# Autodesk Inventor assembly: rodAndKey
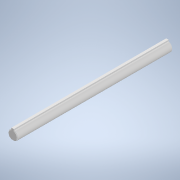
[picture p0: Inventor's stored thumbnail of the model, 180x180]
Saved by Autodesk Inventor 2020.2 (Build 242310000, 310)
## iProperties
Created: 2019-12-09
Part Number: rodAndKey
Document SubType Name: Assembly
Designer: robst
Author: robst
## Documents named in this file (3)
- C:\git\CAD-Development\robSteele\liftSpool\rodAndKey.iam
- C:\git\CAD-Development\robSteele\liftSpool\6 inch 98491A098_OVERSIZED STEEL MACHINE KEY STOCK.ipt
- C:\git\CAD-Development\robSteele\liftSpool\6 inch 1570K330_FULLY KEYED ALUMINUM DRIVE SHAFT.ipt
## Components (2 placed, 2 different names)
1. 6 inch 1570K330_FULLY KEYED ALUMINUM DRIVE SHAFT:1
2. 6 inch 98491A098_OVERSIZED STEEL MACHINE KEY STOCK:1
## Relationships (2: Mate 1, Flush 1)
- [Mate]: 6 inch 1570K330_FULLY KEYED ALUMINUM DRIVE SHAFT:1 ↔ 6 inch 98491A098_OVERSIZED STEEL MACHINE KEY STOCK:1
- [Flush]: 6 inch 1570K330_FULLY KEYED ALUMINUM DRIVE SHAFT:1 ↔ 6 inch 98491A098_OVERSIZED STEEL MACHINE KEY STOCK:1
